# Autodesk Inventor assembly: Roda
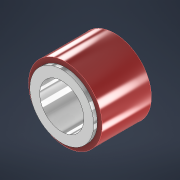
[picture p0: Inventor's stored thumbnail of the model, 180x180]
Saved by Autodesk Inventor 2021 (Build 250183000, 183)
## iProperties
Created: 2021-02-02
Part Number: Roda
Document SubType Name: Assembly
Designer: João
Author: João
## Documents named in this file (4)
- C:\Users\João\Documents\Inventor\SumoCar\GearMotor\Roda.iam
- C:\Users\João\Documents\Inventor\SumoCar\GearMotor\Roda - Estrutura.ipt
- C:\Users\João\Documents\Inventor\SumoCar\GearMotor\Roda - Fixador de eixo.ipt
- C:\Users\João\Documents\Inventor\SumoCar\GearMotor\Roda - Pneu.ipt
## Components (3 placed, 3 different names)
1. Roda - Estrutura:1 — Coincidente:1, Coincidente:2, Coincidente:3, Alinhado:1, Ângulo:1, Coincidente:5
2. Roda - Fixador de eixo:1 — Coincidente:1, Coincidente:4
3. Roda - Pneu:1 — Coincidente:2, Coincidente:3, Ângulo:1, Coincidente:5
## Relationships (7: Mate 5, Flush 1, Angle 1)
- Coincidente:1 [Mate]: Roda - Estrutura:1 ↔ Roda - Fixador de eixo:1
- Coincidente:2 [Mate]: Roda - Estrutura:1 ↔ Roda - Pneu:1
- Coincidente:3 [Mate]: Roda - Estrutura:1 ↔ Roda - Pneu:1
- Alinhado:1 [Flush] (-12 mm): Roda - Estrutura:1
- Coincidente:4 [Mate]: Roda - Fixador de eixo:1
- Ângulo:1 [Angle] (0 deg): Roda - Estrutura:1 ↔ Roda - Pneu:1
- Coincidente:5 [Mate]: Roda - Estrutura:1 ↔ Roda - Pneu:1
